# Autodesk Inventor assembly: Charging port
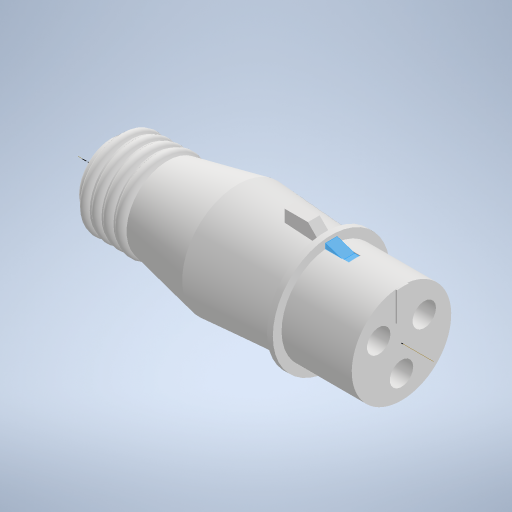
[picture p0: Inventor's stored thumbnail of the model, 512x512]
Saved by Autodesk Inventor 2023 (Build 270158000, 158)
## iProperties
Created: 2023-11-07
Part Number: Charging port
Document SubType Name: Assembly
Designer: Rahul
Author: Rahul
## Documents named in this file (3)
- C:\Users\Rahul\OneDrive\Documents\Charging port.iam
- C:\Users\Rahul\OneDrive\Documents\finalproject2.ipt
- C:\Users\Rahul\OneDrive\Documents\last.ipt
## Components (2 placed, 2 different names)
1. finalproject2:1 — Cylindrical:1, Mate:1
2. last:1 — Cylindrical:1, Mate:1
## Relationships (2: CylindricalJoint 1, Mate 1)
- Cylindrical:1: finalproject2:1 ↔ last:1
- Mate:1: finalproject2:1 ↔ last:1
